# Autodesk Inventor assembly: Silnik
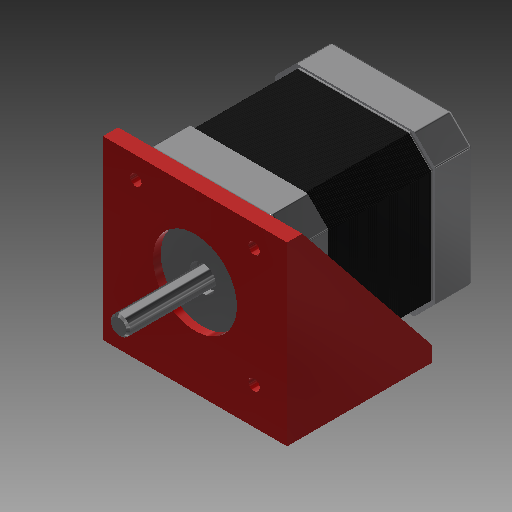
[picture p0: Inventor's stored thumbnail of the model, 512x512]
Saved by Autodesk Inventor 2017 (Build 210142000, 142)
## iProperties
Part Number: Silnik
Material: Ogólny
Document SubType Name: Assembly
Designer: Wojciech
Author: Wojciech
## Documents named in this file (3)
- C:\Users\Wojciech\Documents\Projekty\Balancer\Model 3D\Silnik.iam
- C:\Users\Wojciech\Documents\Projekty\Balancer\Model 3D\NEMA 17.ipt
- C:\Users\Wojciech\Documents\Projekty\Balancer\Model 3D\Ucwyt_NEMA17.ipt
## Components (2 placed, 2 different names)
1. NEMA 17:1 — Zestawiający:1, Zestawiający:2, Zestawiający:3
2. Ucwyt_NEMA17:2 — Zestawiający:1, Zestawiający:2, Zestawiający:3
## Relationships (3: Mate 3)
- Zestawiający:1 [Mate]: NEMA 17:1 ↔ Ucwyt_NEMA17:2
- Zestawiający:2 [Mate]: NEMA 17:1 ↔ Ucwyt_NEMA17:2
- Zestawiający:3 [Mate]: NEMA 17:1 ↔ Ucwyt_NEMA17:2
